# Autodesk Inventor assembly: Full payload assembly with plate
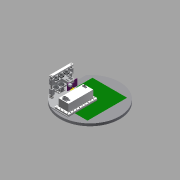
[picture p0: Inventor's stored thumbnail of the model, 180x180]
Saved by Autodesk Inventor 2017 (Build 210142000, 142)
## iProperties
Created: 2016-12-06
Part Number: Full payload assembly with plate
Document SubType Name: Assembly
Designer: qupec
Author: qupec
## Documents named in this file (2)
- C:\Users\qupec\Desktop\UMD Near Space\STAR\CAD\Mechanical\Full payload assembly with plate.iam
- C:\Users\qupec\Desktop\UMD Near Space\STAR\CAD\Mechanical\RockSat Plate.ipt
## Components (2 placed, 2 different names)
1. RockSat Plate:1 — Mate:1, Tangent:1
2. Full payload assembly mk 2:1 [sub-assembly] — Mate:1, Tangent:1
## Relationships (2: Mate 1, Tangent 1)
- Mate:1: RockSat Plate:1 ↔ Full payload assembly mk 2:1
- Tangent:1: RockSat Plate:1 ↔ Full payload assembly mk 2:1
